# Autodesk Inventor assembly: BottomRobot
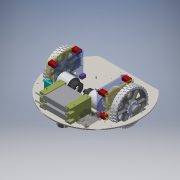
[picture p0: Inventor's stored thumbnail of the model, 180x180]
Saved by Autodesk Inventor 2019 (Build 230136000, 136)
## iProperties
Created: 2020-03-02
Part Number: BottomRobot
Document SubType Name: Assembly
Designer: james
Author: james
## Documents named in this file (15)
- F:\JimsRobot\FIRSTRobots\Design\TornadoPlatypus\BottomRobot.iam
- F:\JimsRobot\FIRSTRobots\Design\TornadoPlatypus\BottomPlate.ipt
- F:\JimsRobot\FIRSTRobots\Design\TornadoPlatypus\MotorLeft.iam
- F:\JimsRobot\FIRSTRobots\Design\TornadoPlatypus\MotorRight.iam
- F:\JimsRobot\FIRSTRobots\Design\Library\Jims\BatteryRail.ipt
- F:\JimsRobot\FIRSTRobots\Design\Library\RevRobotics\REV-31-1302.ipt
- F:\JimsRobot\FIRSTRobots\Design\Library\Fasteners\Size-10-32\HexCap - .5.ipt
- F:\JimsRobot\FIRSTRobots\Design\Library\AndyMark\am-0282 120a Circuit Breaker.ipt
- F:\JimsRobot\FIRSTRobots\Design\Library\SlamTech\RPLIDAR A2.iam
- F:\JimsRobot\FIRSTRobots\Design\Library\Jims\JetsonPlate.ipt
- F:\JimsRobot\FIRSTRobots\Design\Library\NVIDIA\Nano\142-13449-1000-A02_ASM.iam
- F:\JimsRobot\FIRSTRobots\Design\Library\McMaster\SocketScrews\8-32\1in 91251A199_BLACK-OXIDE ALLOY STEEL SOCKET HEAD CAP SCREW.ipt
- F:\JimsRobot\FIRSTRobots\Design\TornadoPlatypus\Slider.iam
- F:\JimsRobot\FIRSTRobots\Design\Library\McMaster\SocketScrews\8-32\3.25in 91251A189_BLACK-OXIDE ALLOY STEEL SOCKET HEAD SCREW.ipt
- F:\JimsRobot\FIRSTRobots\Design\TornadoPlatypus\PowerPlugBlock.iam
## Components (21 placed, 14 different names)
1. BottomPlate:1 — Mate:1, Mate:2, Mate:3, Mate:4, Mate:5, Mate:6, Mate:7, Mate:10, Mate:11, Mate:12, Mate:43, Mate:44, Mate:45, Mate:46, Mate:47, Mate:48, Mate:49, Mate:50, Mate:54, Mate:56, Mate:59, Mate:61, Mate:63, Mate:64, Mate:65, Mate:66, Mate:67, Mate:69, Mate:70, Mate:71, Mate:72, Mate:77, Mate:78, Mate:79
2. MotorLeft:1 [sub-assembly] — Mate:1, Mate:3, Mate:5
3. MotorRight:1 [sub-assembly] — Mate:2, Mate:4
4. BatteryRail:1 — Mate:6, Mate:7, Mate:9, Flush:1, Flush:2
5. BatteryRail:2 — Mate:10, Mate:11, Mate:12, Mate:13, Flush:3, Flush:4, Mate:14, Mate:15
6. BatteryRail:3 — Mate:9, Flush:1, Flush:2, Mate:16, Mate:17
7. BatteryRail:4 — Mate:13, Flush:3, Flush:4
8. REV-31-1302:1 — Mate:14, Mate:15
9. REV-31-1302:2 — Mate:16, Mate:17
10. am-0282 120a Circuit Breaker:1 — Mate:43, Mate:44
11. RPLIDAR A2:1 [sub-assembly] — Mate:45, Mate:46, Mate:47
12. JetsonPlate:1 — Mate:48, Mate:49, Mate:50, Mate:51, Mate:52, Mate:53
13. 142-13449-1000-A02_ASM:1 [sub-assembly] — Mate:51, Mate:52, Mate:53
14. HexCap - .5:6 — Mate:56, Mate:59
15. HexCap - .5:8 — Mate:54, Mate:61
16. 1in 91251A199_BLACK-OXIDE ALLOY STEEL SOCKET HEAD CAP SCREW:1 — Mate:65, Mate:67
17. 1in 91251A199_BLACK-OXIDE ALLOY STEEL SOCKET HEAD CAP SCREW:2 — Mate:64, Mate:66
18. 1in 91251A199_BLACK-OXIDE ALLOY STEEL SOCKET HEAD CAP SCREW:3 — Mate:63, Mate:69
19. Slider:1 [sub-assembly] — Mate:70, Mate:71, Mate:72, Mate:75, Mate:76
20. 3.25in 91251A189_BLACK-OXIDE ALLOY STEEL SOCKET HEAD SCREW:1 — Mate:75, Mate:76
21. PowerPlugBlock:1 [sub-assembly] — Mate:77, Mate:78, Mate:79
## Relationships (49: Mate 45, Flush 4)
- Mate:1: BottomPlate:1 ↔ MotorLeft:1
- Mate:2: BottomPlate:1 ↔ MotorRight:1
- Mate:3: BottomPlate:1 ↔ MotorLeft:1
- Mate:4: BottomPlate:1 ↔ MotorRight:1
- Mate:5: BottomPlate:1 ↔ MotorLeft:1
- Mate:6: BottomPlate:1 ↔ BatteryRail:1
- Mate:7: BottomPlate:1 ↔ BatteryRail:1
- Mate:9: BatteryRail:1 ↔ BatteryRail:3
- Flush:1: BatteryRail:1 ↔ BatteryRail:3
- Flush:2: BatteryRail:1 ↔ BatteryRail:3
- Mate:10: BottomPlate:1 ↔ BatteryRail:2
- Mate:11: BottomPlate:1 ↔ BatteryRail:2
- Mate:12: BottomPlate:1 ↔ BatteryRail:2
- Mate:13: BatteryRail:2 ↔ BatteryRail:4
- Flush:3: BatteryRail:2 ↔ BatteryRail:4
- Flush:4: BatteryRail:2 ↔ BatteryRail:4
- Mate:14: BatteryRail:2 ↔ REV-31-1302:1
- Mate:15: BatteryRail:2 ↔ REV-31-1302:1
- Mate:16: BatteryRail:3 ↔ REV-31-1302:2
- Mate:17: BatteryRail:3 ↔ REV-31-1302:2
- Mate:43: BottomPlate:1 ↔ am-0282 120a Circuit Breaker:1
- Mate:44: BottomPlate:1 ↔ am-0282 120a Circuit Breaker:1
- Mate:45: BottomPlate:1 ↔ RPLIDAR A2:1
- Mate:46: BottomPlate:1 ↔ RPLIDAR A2:1
- Mate:47: BottomPlate:1 ↔ RPLIDAR A2:1
- Mate:48: BottomPlate:1 ↔ JetsonPlate:1
- Mate:49: BottomPlate:1 ↔ JetsonPlate:1
- Mate:50: BottomPlate:1 ↔ JetsonPlate:1
- Mate:51: JetsonPlate:1 ↔ 142-13449-1000-A02_ASM:1
- Mate:52: JetsonPlate:1 ↔ 142-13449-1000-A02_ASM:1
- Mate:53: JetsonPlate:1 ↔ 142-13449-1000-A02_ASM:1
- Mate:54: BottomPlate:1 ↔ HexCap - .5:8
- Mate:56: BottomPlate:1 ↔ HexCap - .5:6
- Mate:59: BottomPlate:1 ↔ HexCap - .5:6
- Mate:61: BottomPlate:1 ↔ HexCap - .5:8
- Mate:63: BottomPlate:1 ↔ 1in 91251A199_BLACK-OXIDE ALLOY STEEL SOCKET HEAD CAP SCREW:3
- Mate:64: BottomPlate:1 ↔ 1in 91251A199_BLACK-OXIDE ALLOY STEEL SOCKET HEAD CAP SCREW:2
- Mate:65: BottomPlate:1 ↔ 1in 91251A199_BLACK-OXIDE ALLOY STEEL SOCKET HEAD CAP SCREW:1
- Mate:66: BottomPlate:1 ↔ 1in 91251A199_BLACK-OXIDE ALLOY STEEL SOCKET HEAD CAP SCREW:2
- Mate:67: BottomPlate:1 ↔ 1in 91251A199_BLACK-OXIDE ALLOY STEEL SOCKET HEAD CAP SCREW:1
- Mate:69: BottomPlate:1 ↔ 1in 91251A199_BLACK-OXIDE ALLOY STEEL SOCKET HEAD CAP SCREW:3
- Mate:70: BottomPlate:1 ↔ Slider:1
- Mate:71: BottomPlate:1 ↔ Slider:1
- Mate:72: BottomPlate:1 ↔ Slider:1
- Mate:75: Slider:1 ↔ 3.25in 91251A189_BLACK-OXIDE ALLOY STEEL SOCKET HEAD SCREW:1
- Mate:76: Slider:1 ↔ 3.25in 91251A189_BLACK-OXIDE ALLOY STEEL SOCKET HEAD SCREW:1
- Mate:77: BottomPlate:1 ↔ PowerPlugBlock:1
- Mate:78: BottomPlate:1 ↔ PowerPlugBlock:1
- Mate:79: BottomPlate:1 ↔ PowerPlugBlock:1
